# Autodesk Inventor assembly: High Strength Chain Generator
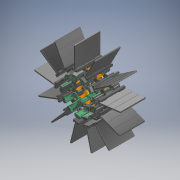
[picture p0: Inventor's stored thumbnail of the model, 180x180]
Saved by Autodesk Inventor 2022 (Build 260153000, 153)
## iProperties
Created: 2020-07-07
Part Number: High Strength Chain Generator
Document SubType Name: Assembly
Designer: yuany
RuleStatus: InUse
AfterDocOpen0: Open Form
Author: yuany
## iProperties of the stored document MemberDocs/xAaaaqbcaAaaaaaaaAaaaqxjcCb
RuleStatus: InUse
Created: 2020-07-07
Part Number: High Strength Chain Generator
Document SubType Name: Assembly
Designer: yuany
AfterDocOpen0: Open Form
Author: yuany
## Documents named in this file (9)
- C:\the7dorks.github.io\Library 1.2\Motion\Chain + Tank Tread\Parametric\High Strength Chain Generator.iam
- C:\the7dorks.github.io\Library 1.2\Motion\Chain + Tank Tread\Parametric\Workpoint Pattern.ipt
- C:\the7dorks.github.io\Library 1.2\Motion\Chain + Tank Tread\High Strength Chain Link.ipt
- C:\the7dorks.github.io\Library 1.2\Motion\Chain + Tank Tread\Tank Tread Traction Link.ipt
- C:\the7dorks.github.io\Library 1.2\Motion\Chain + Tank Tread\Tread Link.ipt
- C:\the7dorks.github.io\Library 1.2\Motion\Chain + Tank Tread\Chain Attachment Link.ipt
- C:\the7dorks.github.io\Library 1.2\Motion\Chain + Tank Tread\Short Flap.ipt
- C:\the7dorks.github.io\Library 1.2\Motion\Chain + Tank Tread\Medium Flap.ipt
- C:\the7dorks.github.io\Library 1.2\Motion\Chain + Tank Tread\Tall Flap.ipt
## Components (92 placed, 8 different names)
1. Workpoint Pattern:3 — Mate:1, Mate:2, Mate:3
2. High Strength Chain Link:1 — Mate:1, Mate:2, Mate:3, Flush:1, Mate:4, Angle:1
3. High Strength Chain Link:2
4. High Strength Chain Link:3
5. High Strength Chain Link:4
6. High Strength Chain Link:5
7. High Strength Chain Link:6
8. High Strength Chain Link:7
9. High Strength Chain Link:8
10. High Strength Chain Link:9
11. High Strength Chain Link:10
12. High Strength Chain Link:11
13. High Strength Chain Link:12
14. High Strength Chain Link:13
15. Tank Tread Traction Link:1 — Flush:1, Mate:4, Angle:1, Flush:2, Mate:5, Angle:2
16. Tank Tread Traction Link:2
17. Tank Tread Traction Link:3
18. Tank Tread Traction Link:4
19. Tank Tread Traction Link:5
20. Tank Tread Traction Link:6
21. Tank Tread Traction Link:7
22. Tank Tread Traction Link:8
23. Tank Tread Traction Link:9
24. Tank Tread Traction Link:10
25. Tank Tread Traction Link:11
26. Tank Tread Traction Link:12
27. Tank Tread Traction Link:13
28. Tread Link:1 — Flush:2, Mate:5, Angle:2, Flush:3, Mate:6, Angle:3
29. Tread Link:2
30. Tread Link:3
31. Tread Link:4
32. Tread Link:5
33. Tread Link:6
34. Tread Link:7
35. Tread Link:8
36. Tread Link:9
37. Tread Link:10
38. Tread Link:11
39. Tread Link:12
40. Tread Link:13
41. Chain Attachment Link:1 — Flush:3, Mate:6, Angle:3
42. Chain Attachment Link:2
43. Chain Attachment Link:3
44. Chain Attachment Link:4
45. Chain Attachment Link:5
46. Chain Attachment Link:6
47. Chain Attachment Link:7
48. Chain Attachment Link:8
49. Chain Attachment Link:9
50. Chain Attachment Link:10
51. Chain Attachment Link:11
52. Chain Attachment Link:12
53. Chain Attachment Link:13
54. Short Flap:1 [sub-assembly]
55. Short Flap:2 [sub-assembly]
56. Short Flap:3 [sub-assembly]
57. Short Flap:4 [sub-assembly]
58. Short Flap:5 [sub-assembly]
59. Short Flap:6 [sub-assembly]
60. Short Flap:7 [sub-assembly]
61. Short Flap:8 [sub-assembly]
62. Short Flap:9 [sub-assembly]
63. Short Flap:10 [sub-assembly]
64. Short Flap:11 [sub-assembly]
65. Short Flap:12 [sub-assembly]
66. Short Flap:13 [sub-assembly]
67. Medium Flap:1 [sub-assembly]
68. Medium Flap:2 [sub-assembly]
69. Medium Flap:3 [sub-assembly]
70. Medium Flap:4 [sub-assembly]
71. Medium Flap:5 [sub-assembly]
72. Medium Flap:6 [sub-assembly]
73. Medium Flap:7 [sub-assembly]
74. Medium Flap:8 [sub-assembly]
75. Medium Flap:9 [sub-assembly]
76. Medium Flap:10 [sub-assembly]
77. Medium Flap:11 [sub-assembly]
78. Medium Flap:12 [sub-assembly]
79. Medium Flap:13 [sub-assembly]
80. Tall Flap:1 [sub-assembly]
81. Tall Flap:2 [sub-assembly]
82. Tall Flap:3 [sub-assembly]
83. Tall Flap:4 [sub-assembly]
84. Tall Flap:5 [sub-assembly]
85. Tall Flap:6 [sub-assembly]
86. Tall Flap:7 [sub-assembly]
87. Tall Flap:8 [sub-assembly]
88. Tall Flap:9 [sub-assembly]
89. Tall Flap:10 [sub-assembly]
90. Tall Flap:11 [sub-assembly]
91. Tall Flap:12 [sub-assembly]
92. Tall Flap:13 [sub-assembly]
## Component patterns: Chain (13 elements), Traction (13 elements), Tread (13 elements), Chain Attachment (13 elements), Short Flaps (13 elements), Medium Flaps (13 elements), Tall Flaps (13 elements)
## Relationships (12: Mate 6, Flush 3, Angle 3)
- Mate:1: Workpoint Pattern:3 ↔ High Strength Chain Link:1
- Mate:2 (11.938 mm): Workpoint Pattern:3 ↔ High Strength Chain Link:1
- Mate:3: Workpoint Pattern:3 ↔ High Strength Chain Link:1
- Flush:1: High Strength Chain Link:1 ↔ Tank Tread Traction Link:1
- Mate:4: High Strength Chain Link:1 ↔ Tank Tread Traction Link:1
- Angle:1 (180 deg): High Strength Chain Link:1 ↔ Tank Tread Traction Link:1
- Flush:2: Tank Tread Traction Link:1 ↔ Tread Link:1
- Mate:5: Tank Tread Traction Link:1 ↔ Tread Link:1
- Angle:2 (0 deg): Tank Tread Traction Link:1 ↔ Tread Link:1
- Flush:3: Tread Link:1 ↔ Chain Attachment Link:1
- Mate:6: Tread Link:1 ↔ Chain Attachment Link:1
- Angle:3 (0 deg): Tread Link:1 ↔ Chain Attachment Link:1
## Named parameters: Center_Distance = 88.9 mm, Sprocket1 = 37.846 mm, Sprocket2 = 37.846 mm, CenterDistance = 0 mm, d5_1 = 0 mm, d6_1 = 0 mm, d7_1 = 59.44836 mm, d8_1 = 59.44836 mm
